# Autodesk Inventor assembly: DriveTrainMotor+MountB
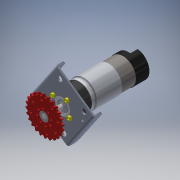
[picture p0: Inventor's stored thumbnail of the model, 180x180]
Saved by Autodesk Inventor 2018 (Build 220112000, 112)
## iProperties
Created: 2017-11-14
Part Number: DriveTrainMotor+MountB
Document SubType Name: Assembly
Designer: ball
Author: ball
## Documents named in this file (6)
- C:\FTC\2017Robot\DriveTrainMotor+MountB.iam
- C:\FTC\Andymark\am-3461a+NeveRest+Orbital+3.7+REV2.ipt
- C:\FTC\Actobotics\615 parts\615106.ipt
- C:\FTC\Actobotics\545 parts\545618 assembly.ipt
- C:\FTC\StepLibraries\Screws\M3x6 SHCS.ipt
- C:\FTC\Andymark\am-3474 drive train mount.ipt
## Components (8 placed, 5 different names)
1. am-3461a+NeveRest+Orbital+3.7+REV2:1 — Mate:16, Flush:1, Flush:2
2. am-3474 drive train mount:2
3. M3x6 SHCS:1
4. M3x6 SHCS:2
5. M3x6 SHCS:3
6. M3x6 SHCS:4
7. 615106:2 — Mate:13, Mate:14, Mate:15
8. 545618 assembly:2 — Mate:13, Mate:14, Mate:15, Mate:16, Flush:1, Flush:2
## Relationships (18: Mate 16, Flush 2)
- [Mate]: am-3461a+NeveRest+Orbital+3.7+REV2:1 ↔ am-3474 drive train mount:2
- [Mate]: am-3461a+NeveRest+Orbital+3.7+REV2:1 ↔ am-3474 drive train mount:2
- [Mate]: am-3461a+NeveRest+Orbital+3.7+REV2:1 ↔ am-3474 drive train mount:2
- [Mate]: am-3461a+NeveRest+Orbital+3.7+REV2:1 ↔ am-3474 drive train mount:2
- [Mate]: am-3474 drive train mount:2 ↔ M3x6 SHCS:4
- [Mate]: am-3474 drive train mount:2 ↔ M3x6 SHCS:3
- [Mate]: am-3474 drive train mount:2 ↔ M3x6 SHCS:1
- [Mate]: am-3474 drive train mount:2 ↔ M3x6 SHCS:2
- [Mate]: am-3474 drive train mount:2 ↔ M3x6 SHCS:4
- [Mate]: am-3474 drive train mount:2 ↔ M3x6 SHCS:1
- [Mate]: am-3474 drive train mount:2 ↔ M3x6 SHCS:3
- [Mate]: am-3474 drive train mount:2 ↔ M3x6 SHCS:2
- Mate:13: 615106:2 ↔ 545618 assembly:2
- Mate:14: 615106:2 ↔ 545618 assembly:2
- Mate:15: 615106:2 ↔ 545618 assembly:2
- Mate:16: am-3461a+NeveRest+Orbital+3.7+REV2:1 ↔ 545618 assembly:2
- Flush:1: am-3461a+NeveRest+Orbital+3.7+REV2:1 ↔ 545618 assembly:2
- Flush:2: am-3461a+NeveRest+Orbital+3.7+REV2:1 ↔ 545618 assembly:2
